# Autodesk Inventor assembly: Model-1
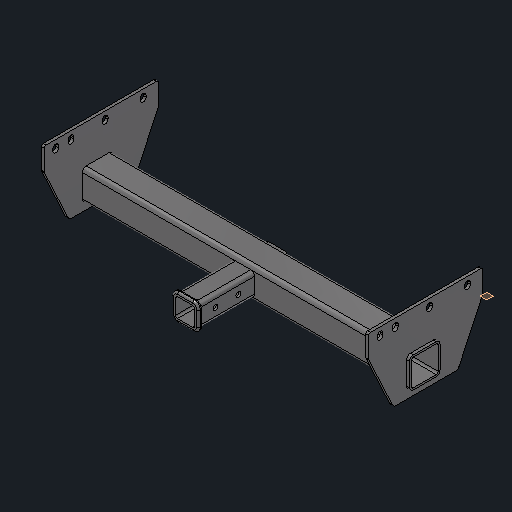
[picture p0: Inventor's stored thumbnail of the model, 512x512]
Saved by Autodesk Inventor 2025.1 (Build 291241000, 241)
## iProperties
Created: 2026-02-13
Part Number: Model-1
Document SubType Name: Assembly
Designer: Desktop -24
encoded128: ÌStandard (in)rÎ
Family: ASSEMBLY
Author: Desktop -24
## Documents named in this file (5)
- F:\OneDrive - nLeague Technologies Private Limited\Desktop\Sharath Chandra\Front Hitch\Front Hitch Model-1\Front Hitch Model-1.iam
- F:\OneDrive - nLeague Technologies Private Limited\Desktop\Sharath Chandra\Front Hitch\Front Hitch Model-1\Front Hitch Model-1_Base Tube-1.ipt
- F:\OneDrive - nLeague Technologies Private Limited\Desktop\Sharath Chandra\Front Hitch\Front Hitch Model-1\Front Hitch Model-1_Base Tube-2.ipt
- F:\OneDrive - nLeague Technologies Private Limited\Desktop\Sharath Chandra\Front Hitch\Front Hitch Model-1\Front Hitch Model-1_Sheet-RH.ipt
- F:\OneDrive - nLeague Technologies Private Limited\Desktop\Sharath Chandra\Front Hitch\Front Hitch Model-1\Front Hitch Model-1_Sheet-LH.ipt
## Components (4 placed, 4 different names)
1. Front Hitch Model-1_Base Tube-1:1 — Mate:14, Mate:15, Mate:16, Mate:17, Mate:18, Flush:8, Flush:9
2. Front Hitch Model-1_Base Tube-2:1
3. Front Hitch Model-1_Sheet-LH:1 — Mate:17, Mate:18, Flush:8
4. Front Hitch Model-1_Sheet-RH:1 — Mate:15, Mate:16, Flush:9
## Relationships (10: Mate 7, Flush 3)
- [Mate]: Front Hitch Model-1_Base Tube-1:1 ↔ Front Hitch Model-1_Base Tube-2:1
- [Mate]: Front Hitch Model-1_Base Tube-1:1 ↔ Front Hitch Model-1_Base Tube-2:1
- [Flush] (9.525 mm): Front Hitch Model-1_Base Tube-1:1 ↔ Front Hitch Model-1_Base Tube-2:1
- Mate:14: Front Hitch Model-1_Base Tube-1:1
- Mate:15: Front Hitch Model-1_Base Tube-1:1 ↔ Front Hitch Model-1_Sheet-RH:1
- Mate:16: Front Hitch Model-1_Base Tube-1:1 ↔ Front Hitch Model-1_Sheet-RH:1
- Mate:17: Front Hitch Model-1_Base Tube-1:1 ↔ Front Hitch Model-1_Sheet-LH:1
- Mate:18: Front Hitch Model-1_Base Tube-1:1 ↔ Front Hitch Model-1_Sheet-LH:1
- Flush:8 (9.525 mm): Front Hitch Model-1_Base Tube-1:1 ↔ Front Hitch Model-1_Sheet-LH:1
- Flush:9 (-9.525 mm): Front Hitch Model-1_Base Tube-1:1 ↔ Front Hitch Model-1_Sheet-RH:1
## Named parameters: d21_d8 = 0 mm, d23_d10 = 9.525 mm
